# Autodesk Inventor assembly: segment1
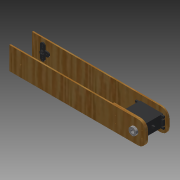
[picture p0: Inventor's stored thumbnail of the model, 180x180]
Saved by Autodesk Inventor 2013 (Build 170138000, 138)
## iProperties
Created: 2014-10-10
Part Number: segment1
Document SubType Name: Assembly
Designer: Masta
Mass: 275.721 g
Surface Area: 991.467 cm^2
Volume: 320.879 cm^3
Density: 0.859269 g/cm^3
Author: Masta
## Documents named in this file (7)
- D:\DrOctopus\3D model\arm\segment1.iam
- D:\DrOctopus\3D model\arm\segment1a.ipt
- D:\DrOctopus\3D model\arm\servo 33kg TGY-S8166M.ipt
- D:\DrOctopus\3D model\arm\servo arm BMS-630MG tripple.ipt
- D:\DrOctopus\3D model\arm\segment1b.ipt
- D:\DrOctopus\3D model\arm\segment1c.ipt
- D:\DrOctopus\3D model\arm\Bearing 699ZZ - 9x20x6mm.ipt
## Components (6 placed, 6 different names)
1. segment1a:2 — Insert:4, Insert:5, Insert:6, Insert:7, Mate:1, Flush:1, Flush:2
2. servo 33kg TGY-S8166M:1 — Insert:6, Insert:7, Insert:10
3. servo arm BMS-630MG tripple:1 — Insert:4, Insert:5
4. segment1b:1 — Insert:8, Insert:9, Mate:1, Flush:1, Flush:2, Mate:2
5. segment1c:1 — Insert:8, Insert:9
6. Bearing 699ZZ - 9x20x6mm:1 — Insert:10, Mate:2
## Relationships (11: Insert 7, Mate 2, Flush 2)
- Insert:4: segment1a:2 ↔ servo arm BMS-630MG tripple:1
- Insert:5: segment1a:2 ↔ servo arm BMS-630MG tripple:1
- Insert:6 (2 mm): segment1a:2 ↔ servo 33kg TGY-S8166M:1
- Insert:7 (2 mm): segment1a:2 ↔ servo 33kg TGY-S8166M:1
- Insert:8: segment1b:1 ↔ segment1c:1
- Insert:9: segment1b:1 ↔ segment1c:1
- Mate:1 (56.5 mm): segment1a:2 ↔ segment1b:1
- Flush:1: segment1a:2 ↔ segment1b:1
- Flush:2: segment1a:2 ↔ segment1b:1
- Insert:10: servo 33kg TGY-S8166M:1 ↔ Bearing 699ZZ - 9x20x6mm:1
- Mate:2: segment1b:1 ↔ Bearing 699ZZ - 9x20x6mm:1
